# Autodesk Inventor assembly: Funnel Plate Assembly
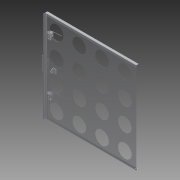
[picture p0: Inventor's stored thumbnail of the model, 180x180]
Saved by Autodesk Inventor 2014 (Build 180170000, 170)
## iProperties
Created: 2014-01-05
Part Number: Funnel Plate Assembly
Document SubType Name: Assembly
Designer: Michael
Mass: 414.636 g
Surface Area: 4954.67 cm^2
Volume: 219.366 cm^3
Density: 1.89016 g/cm^3
Author: Michael
## Documents named in this file (6)
- C:\Users\Michael\Documents\Robotics\2014 Season\Funnel Catcher\Funnel Plate Assembly.iam
- C:\Users\Michael\Documents\Robotics\2014 Season\Funnel Catcher\Plastic Funnel PIece.ipt
- C:\Users\Michael\Documents\Robotics\2014 Season\Funnel Catcher\.05 in Aluminum Angle.ipt
- C:\Users\Michael\Documents\Robotics\2014 Season\Funnel Catcher\Flange for Torsion Spring.ipt
- C:\Users\Michael\Documents\Robotics\2014 Season\Funnel Catcher\360 degree Torsion Spring (9271K134).ipt
- C:\Users\Michael\Documents\Robotics\2014 Season\Funnel Catcher\Piano Hinge (15665A319).ipt
## Components (12 placed, 5 different names)
1. Plastic Funnel PIece:1 — Insert:25, Insert:26, Angle:1, Angle:2, Insert:51, Insert:52, Insert:53, Insert:54, Insert:55, Insert:56, Insert:57, Insert:58, Insert:59, Insert:60, Insert:61, Insert:62, Insert:63, Insert:64, Insert:65, Insert:66
2. .05 in Aluminum Angle:1 — Insert:25, Insert:26
3. Flange for Torsion Spring:2 — Insert:59, Insert:60
4. Flange for Torsion Spring:4 — Insert:56, Insert:57
5. Flange for Torsion Spring:5 — Mate:2, Mate:4, Insert:61, Insert:62
6. Flange for Torsion Spring:7 — Mate:1, Mate:3, Insert:55, Insert:58
7. 360 degree Torsion Spring (9271K134):1 — Mate:2, Angle:2, Mate:4
8. 360 degree Torsion Spring (9271K134):2 — Mate:1, Angle:1, Mate:3
9. .05 in Aluminum Angle:3 — Insert:51, Insert:52
10. .05 in Aluminum Angle:4 — Insert:53, Insert:54
11. Piano Hinge (15665A319):1 — Insert:63, Insert:64
12. Flange for Torsion Spring:8 — Insert:65, Insert:66
## Relationships (24: Insert 18, Mate 4, Angle 2)
- Insert:25: Plastic Funnel PIece:1 ↔ .05 in Aluminum Angle:1
- Insert:26: Plastic Funnel PIece:1 ↔ .05 in Aluminum Angle:1
- Mate:1: Flange for Torsion Spring:7 ↔ 360 degree Torsion Spring (9271K134):2
- Mate:2: Flange for Torsion Spring:5 ↔ 360 degree Torsion Spring (9271K134):1
- Angle:1 (90 deg): Plastic Funnel PIece:1 ↔ 360 degree Torsion Spring (9271K134):2
- Angle:2 (90 deg): Plastic Funnel PIece:1 ↔ 360 degree Torsion Spring (9271K134):1
- Mate:3 (4.7625 mm): Flange for Torsion Spring:7 ↔ 360 degree Torsion Spring (9271K134):2
- Mate:4 (4.7625 mm): Flange for Torsion Spring:5 ↔ 360 degree Torsion Spring (9271K134):1
- Insert:51: Plastic Funnel PIece:1 ↔ .05 in Aluminum Angle:3
- Insert:52: Plastic Funnel PIece:1 ↔ .05 in Aluminum Angle:3
- Insert:53: Plastic Funnel PIece:1 ↔ .05 in Aluminum Angle:4
- Insert:54: Plastic Funnel PIece:1 ↔ .05 in Aluminum Angle:4
- Insert:55: Plastic Funnel PIece:1 ↔ Flange for Torsion Spring:7
- Insert:56: Plastic Funnel PIece:1 ↔ Flange for Torsion Spring:4
- Insert:57: Plastic Funnel PIece:1 ↔ Flange for Torsion Spring:4
- Insert:58: Plastic Funnel PIece:1 ↔ Flange for Torsion Spring:7
- Insert:59: Plastic Funnel PIece:1 ↔ Flange for Torsion Spring:2
- Insert:60: Plastic Funnel PIece:1 ↔ Flange for Torsion Spring:2
- Insert:61: Plastic Funnel PIece:1 ↔ Flange for Torsion Spring:5
- Insert:62: Plastic Funnel PIece:1 ↔ Flange for Torsion Spring:5
- Insert:63: Plastic Funnel PIece:1 ↔ Piano Hinge (15665A319):1
- Insert:64: Plastic Funnel PIece:1 ↔ Piano Hinge (15665A319):1
- Insert:65: Plastic Funnel PIece:1 ↔ Flange for Torsion Spring:8
- Insert:66: Plastic Funnel PIece:1 ↔ Flange for Torsion Spring:8
